# Autodesk Inventor assembly: _TOP
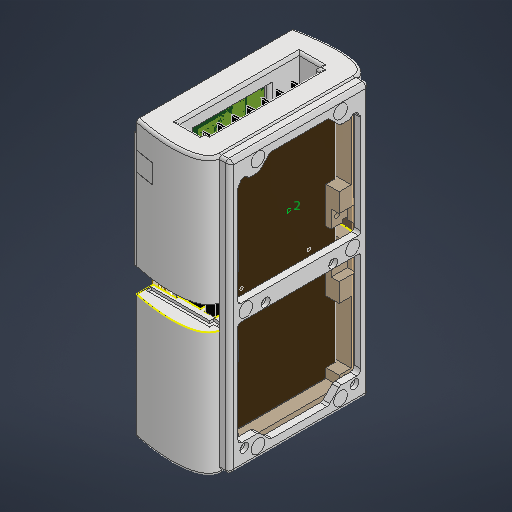
[picture p0: Inventor's stored thumbnail of the model, 512x512]
Saved by Autodesk Inventor 2026.1 (Build 301233020, 233B)
## iProperties
Created: 2025-09-11
Part Number: _TOP
Document SubType Name: Assembly
Designer: atrus
Author: atrus
## Documents named in this file (11)
- C:\Users\atrus\Dropbox\elec\Mechanical\LEDBrick\_TOP.iam
- C:\Users\atrus\Dropbox\elec\Mechanical\LEDBrick\HeatSink3.5.ipt
- C:\Users\atrus\Dropbox\elec\Mechanical\LEDBrick\PCB\rv_ledbrick_8ch.iam
- C:\Users\atrus\Dropbox\elec\Mechanical\LEDBrick\NF-A9x14 PWM\NF-A9x14 PWM\NF-A9x14 PWM.iam
- C:\Users\atrus\Dropbox\elec\Mechanical\LEDBrick\BP_FrontHSCover.ipt
- C:\Users\atrus\Dropbox\elec\Mechanical\LEDBrick\BP_BackHSCover.ipt
- C:\Users\atrus\Dropbox\elec\Mechanical\LEDBrick\BP_Center.ipt
- C:\Users\atrus\Dropbox\elec\Mechanical\LEDBrick\BP_CoverPlateAcrylic.ipt
- C:\Users\atrus\Dropbox\elec\Mechanical\LEDBrick\BP_ShroudAdapter.ipt
- C:\Users\atrus\Dropbox\elec\Mechanical\LEDBrick\BP_FanCover.ipt
- C:\Users\atrus\Dropbox\elec\Mechanical\LEDBrick\BP_BackCover.ipt
## Components (10 placed, 10 different names)
1. HeatSink3.5:1 — Flush:1, Mate:1, Mate:2, Mate:3, Mate:4, Flush:2, Flush:3, Flush:4, Flush:5, Flush:6, Flush:7
2. rv_ledbrick_8ch:1 [sub-assembly] — Mate:1, Mate:2, Flush:2
3. NF-A9x14 PWM:2 [sub-assembly] — Flush:1, Mate:3, Mate:4
4. BP_FrontHSCover:1 — Flush:3, Flush:4, Flush:12, Flush:13
5. BP_BackHSCover:1 — Flush:5, Flush:6, Flush:7, Flush:8, Flush:9, Flush:14, Flush:15
6. BP_Center:1 — Flush:8, Flush:9, Mate:5
7. BP_CoverPlateAcrylic:1 — Mate:5, Flush:10, Flush:11
8. BP_ShroudAdapter:1 — Flush:10, Flush:11
9. BP_FanCover:1 — Flush:12, Flush:13
10. BP_BackCover:1 — Flush:14, Flush:15
## Relationships (20: Flush 15, Mate 5)
- Flush:1: HeatSink3.5:1 ↔ NF-A9x14 PWM:2
- Mate:1 (-5 mm): HeatSink3.5:1 ↔ rv_ledbrick_8ch:1
- Mate:2: HeatSink3.5:1 ↔ rv_ledbrick_8ch:1
- Mate:3: HeatSink3.5:1 ↔ NF-A9x14 PWM:2
- Mate:4: HeatSink3.5:1 ↔ NF-A9x14 PWM:2
- Flush:2 (-5 mm): HeatSink3.5:1 ↔ rv_ledbrick_8ch:1
- Flush:3: HeatSink3.5:1 ↔ BP_FrontHSCover:1
- Flush:4: HeatSink3.5:1 ↔ BP_FrontHSCover:1
- Flush:5: HeatSink3.5:1 ↔ BP_BackHSCover:1
- Flush:6: HeatSink3.5:1 ↔ BP_BackHSCover:1
- Flush:7 (0.2 mm): HeatSink3.5:1 ↔ BP_BackHSCover:1
- Flush:8: BP_BackHSCover:1 ↔ BP_Center:1
- Flush:9: BP_BackHSCover:1 ↔ BP_Center:1
- Mate:5: BP_Center:1 ↔ BP_CoverPlateAcrylic:1
- Flush:10: BP_CoverPlateAcrylic:1 ↔ BP_ShroudAdapter:1
- Flush:11: BP_CoverPlateAcrylic:1 ↔ BP_ShroudAdapter:1
- Flush:12: BP_FrontHSCover:1 ↔ BP_FanCover:1
- Flush:13: BP_FrontHSCover:1 ↔ BP_FanCover:1
- Flush:14: BP_BackHSCover:1 ↔ BP_BackCover:1
- Flush:15: BP_BackHSCover:1 ↔ BP_BackCover:1
